# Autodesk Inventor assembly: Assembly_Cube
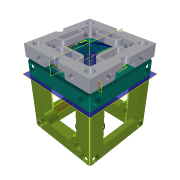
[picture p0: Inventor's stored thumbnail of the model, 180x180]
Saved by Autodesk Inventor 2016 (Build 200138000, 138)
## iProperties
Created: 2018-06-11
Part Number: Assembly_Cube
Material: Generisch
Document SubType Name: Assembly
Designer: diederichbenedict
Author: diederichbenedict
## Documents named in this file (6)
- C:\Users\diederichbenedict\Dropbox\Dokumente\Promotion\PROJECTS\E.COLI\02_CAD\INVENTOR\E.ColiV4\10_Cube_Base\Assembly_Cube.iam
- C:\Users\diederichbenedict\Dropbox\Dokumente\Promotion\PROJECTS\E.COLI\02_CAD\INVENTOR\E.ColiV4\10_Cube_Base\10_Lid_el_v0.ipt
- C:\Users\diederichbenedict\Dropbox\Dokumente\Promotion\PROJECTS\E.COLI\02_CAD\INVENTOR\E.ColiV4\10_Cube_Base\10_Cube_v0.ipt
- C:\Users\diederichbenedict\Dropbox\Dokumente\Promotion\PROJECTS\E.COLI\02_CAD\INVENTOR\E.ColiV4\10_Cube_Base\00_Base_v0.ipt
- C:\Users\diederichbenedict\Dropbox\Dokumente\Promotion\PROJECTS\E.COLI\02_CAD\INVENTOR\E.ColiV4\10_Cube_Base\00_BallMagnets_6mm.ipt
- C:\Users\diederichbenedict\Documents\Inventor\Content Center Files\R2016\de-DE\DIN 912\DIN 912 - M3 x 0.5 x 12 x 10.75.ipt
## Components (8 placed, 5 different names)
1. 10_Lid_el_v0:1 — Einfügen:3, Einfügen:4, Einfügen:5, Einfügen:6, Winkel:1
2. 10_Cube_v0:1
3. 00_Base_v0:1 — Passend:1, Einfügen:7, Winkel:1
4. 00_BallMagnets_6mm:1 — Passend:1
5. DIN 912 - ersetzt durch DIN EN ISO 4762 M3 x 12:1 — Einfügen:4, Einfügen:7
6. DIN 912 - ersetzt durch DIN EN ISO 4762 M3 x 12:2 — Einfügen:3
7. DIN 912 - ersetzt durch DIN EN ISO 4762 M3 x 12:3 — Einfügen:5
8. DIN 912 - ersetzt durch DIN EN ISO 4762 M3 x 12:4 — Einfügen:6
## Relationships (9: Insert 7, Mate 1, Angle 1)
- [Insert]: 10_Lid_el_v0:1 ↔ 10_Cube_v0:1
- [Insert]: 10_Lid_el_v0:1 ↔ 10_Cube_v0:1
- Passend:1 [Mate]: 00_Base_v0:1 ↔ 00_BallMagnets_6mm:1
- Einfügen:3 [Insert]: 10_Lid_el_v0:1 ↔ DIN 912 - ersetzt durch DIN EN ISO 4762 M3 x 12:2
- Einfügen:4 [Insert]: 10_Lid_el_v0:1 ↔ DIN 912 - ersetzt durch DIN EN ISO 4762 M3 x 12:1
- Einfügen:5 [Insert]: 10_Lid_el_v0:1 ↔ DIN 912 - ersetzt durch DIN EN ISO 4762 M3 x 12:3
- Einfügen:6 [Insert]: 10_Lid_el_v0:1 ↔ DIN 912 - ersetzt durch DIN EN ISO 4762 M3 x 12:4
- Einfügen:7 [Insert] (1 mm): 00_Base_v0:1 ↔ DIN 912 - ersetzt durch DIN EN ISO 4762 M3 x 12:1
- Winkel:1 [Angle] (180 deg): 10_Lid_el_v0:1 ↔ 00_Base_v0:1
